# Autodesk Inventor assembly: axis5_6
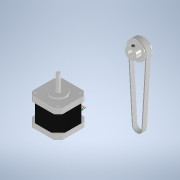
[picture p0: Inventor's stored thumbnail of the model, 180x180]
Saved by Autodesk Inventor 2020 (Build 240168000, 168)
## iProperties
Created: 2020-05-15
Part Number: axis5_6
Document SubType Name: Assembly
Designer: stefa
Author: stefa
## Documents named in this file (4)
- D:\github_gedeeld\BeerMinder\3D-model\axis5_6\axis5_6.iam
- D:\github_gedeeld\BeerMinder\3D-model\pulleys\tandriem32Tnaar16T_lengte240.ipt
- D:\github_gedeeld\BeerMinder\3D-model\pulleys\GT2 Timing Pulley 36T - 8mm as.ipt
- D:\github_gedeeld\BeerMinder\3D-model\stepper motors\42BYG Stepper Motor.ipt
## Components (3 placed, 3 different names)
1. tandriem32Tnaar16T_lengte240:1 — Mate:3, Mate:4
2. GT2 Timing Pulley 36T - 8mm as:1 — Mate:3, Mate:4
3. 42BYG Stepper Motor:1
## Relationships (2: Mate 2)
- Mate:3 (0.5 mm): tandriem32Tnaar16T_lengte240:1 ↔ GT2 Timing Pulley 36T - 8mm as:1
- Mate:4: tandriem32Tnaar16T_lengte240:1 ↔ GT2 Timing Pulley 36T - 8mm as:1
